# Autodesk Inventor assembly: ASY дренаж угольные
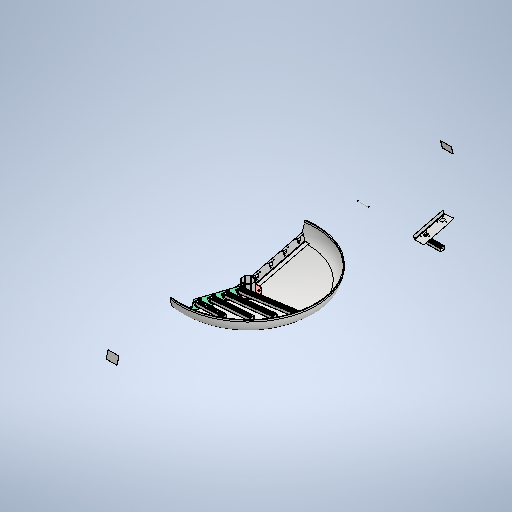
[picture p0: Inventor's stored thumbnail of the model, 512x512]
Saved by Autodesk Inventor 2025.1 (Build 291241020, 241B)
## iProperties
Created: 2024-12-09
Part Number: ASY дренаж угольные
Document SubType Name: Assembly
Designer: user
Author: user
## Documents named in this file (24)
- C:\Users\user\YandexDisk-badmisterfox\home pc\Inventor\filter-distribution-system\ASY BOTTOM filter distribution system.iam
- C:\Users\user\YandexDisk-badmisterfox\home pc\Inventor\filter-distribution-system\drain flange.ipt
- C:\Users\user\YandexDisk-badmisterfox\home pc\Inventor\filter-distribution-system\Фильтр напорный угольный 30 куб час.ipt
- C:\Users\user\YandexDisk-badmisterfox\home pc\Inventor\filter-distribution-system\MNT-CDF-501 box.ipt
- C:\Users\user\YandexDisk-badmisterfox\home pc\Inventor\filter-distribution-system\MNT-CDF-502 tube.ipt
- C:\Users\user\YandexDisk-badmisterfox\home pc\Inventor\filter-distribution-system\MNT-CDF-503  main tube 1.ipt
- C:\Users\user\YandexDisk-badmisterfox\home pc\Inventor\filter-distribution-system\MNT-CDF-504 small tube flange.ipt
- C:\Users\user\YandexDisk-badmisterfox\home pc\Inventor\filter-distribution-system\MNT-CDF-315 beam 5.ipt
- C:\Users\user\YandexDisk-badmisterfox\home pc\Inventor\filter-distribution-system\MNT-CDF-312 beam 2.ipt
- C:\Users\user\YandexDisk-badmisterfox\home pc\Inventor\filter-distribution-system\MNT-CDF-313 beam 3.ipt
- C:\Users\user\YandexDisk-badmisterfox\home pc\Inventor\filter-distribution-system\MNT-CDF-314 beam 4.ipt
- C:\Users\user\YandexDisk-badmisterfox\home pc\Inventor\filter-distribution-system\MNT-CDF-601 CAP.ipt
- C:\Users\user\YandexDisk-badmisterfox\home pc\Inventor\filter-distribution-system\MNT-CDF-602 CAP.ipt
- C:\Users\user\YandexDisk-badmisterfox\home pc\Inventor\filter-distribution-system\MNT-CDF-603 CAP.ipt
- C:\Users\user\YandexDisk-badmisterfox\home pc\Inventor\filter-distribution-system\ASY Луч 1.iam
- C:\Users\user\YandexDisk-badmisterfox\home pc\Inventor\filter-distribution-system\MNT-CDF-402 roof 875.ipt
- C:\Users\user\YandexDisk-badmisterfox\home pc\Inventor\filter-distribution-system\MNT-CDF-403 roof 775.ipt
- C:\Users\user\YandexDisk-badmisterfox\home pc\Inventor\filter-distribution-system\MNT-CDF-404 roof 675.ipt
- C:\Users\user\YandexDisk-badmisterfox\home pc\Inventor\filter-distribution-system\MNT-CDF-405 roof 475.ipt
- C:\Users\user\YandexDisk-badmisterfox\home pc\Inventor\filter-distribution-system\000 DS-B dimentions.ipt
- C:\Users\user\YandexDisk-badmisterfox\home pc\Inventor\filter-distribution-system\000 DS-B outer tube.ipt
- C:\Users\user\YandexDisk-badmisterfox\home pc\Inventor\filter-distribution-system\110 DS-B drain sustem flange.ipt
- C:\Users\user\YandexDisk-badmisterfox\home pc\Inventor\filter-distribution-system\MNT-CDF-613 big way.ipt
- C:\Users\user\YandexDisk-badmisterfox\home pc\Inventor\filter-distribution-system\MNT-CDF-604 CAP.ipt
## Components (34 placed, 23 different names)
1. 000 DS-B dimentions:1
2. Фильтр напорный угольный 30 куб час:1 — Mate:4, Flush:3, Flush:4, Rigid:36
3. MNT-CDF-501 box:1 — Mate:5, Flush:5, Mate:6, Rigid:40, Rigid:42, Rigid:43, Rigid:46, Rigid:47
4. drain flange:2 — Rigid:37
5. MNT-CDF-502 tube:4
6. MNT-CDF-502 tube:3
7. MNT-CDF-502 tube:2
8. MNT-CDF-503  main tube 1:1 — Rigid:39, Mate:7
9. MNT-CDF-503  main tube 1:2 — Mate:5, Rigid:38
10. MNT-CDF-501 box:2 — Mate:7, Mate:8, Mate:9
11. MNT-CDF-502 tube:5
12. MNT-CDF-405 roof 475:1 — Flush:15, Flush:16, Flush:17
13. MNT-CDF-315 beam 5:1 — Rigid:48, Flush:15, Flush:16, Flush:17
14. Part1:5 — Rigid:48
15. MNT-CDF-402 roof 875:1 — Flush:6, Flush:7, Flush:8
16. Part1:6 — Rigid:26, Rigid:43
17. MNT-CDF-604 CAP:1 — Rigid:44
18. MNT-CDF-312 beam 2:1 — Rigid:26, Flush:6, Flush:7, Flush:8, Rigid:44
19. Part1:7 — Rigid:27, Rigid:46
20. Part1:8 — Rigid:28, Rigid:47
21. MNT-CDF-313 beam 3:1 — Rigid:27, Flush:9, Flush:10, Flush:11, Rigid:45
22. MNT-CDF-403 roof 775:1 — Flush:9, Flush:10, Flush:11
23. MNT-CDF-404 roof 675:1 — Flush:12, Flush:13, Flush:14
24. MNT-CDF-314 beam 4:1 — Rigid:28, Flush:12, Flush:13, Flush:14
25. MNT-CDF-601 CAP:1
26. MNT-CDF-602 CAP:1
27. MNT-CDF-602 CAP:2
28. MNT-CDF-603 CAP:1 — Rigid:40, Rigid:41
29. MNT-CDF-603 CAP:2
30. ASY Луч 1:1 [sub-assembly] — Rigid:42
31. 000 DS-B outer tube:1 — Rigid:36, Rigid:37
32. drain sustem flange:1 — Mate:6, Rigid:38, Rigid:39, Mate:8
33. MNT-CDF-613 big way:1 — Rigid:41
34. MNT-CDF-604 CAP:2 — Rigid:45
## Relationships (37: WeldJoint 16, Flush 15, Mate 6)
- Mate:4: Фильтр напорный угольный 30 куб час:1
- Flush:3: Фильтр напорный угольный 30 куб час:1
- Flush:4: Фильтр напорный угольный 30 куб час:1
- Rigid:26 [WeldJoint]: Part1:6 ↔ MNT-CDF-312 beam 2:1
- Rigid:27 [WeldJoint]: Part1:7 ↔ MNT-CDF-313 beam 3:1
- Rigid:28 [WeldJoint]: Part1:8 ↔ MNT-CDF-314 beam 4:1
- Rigid:36 [WeldJoint]: Фильтр напорный угольный 30 куб час:1 ↔ 000 DS-B outer tube:1
- Rigid:37 [WeldJoint]: drain flange:2 ↔ 000 DS-B outer tube:1
- Mate:5: MNT-CDF-501 box:1 ↔ MNT-CDF-503  main tube 1:2
- Flush:5: MNT-CDF-501 box:1
- Mate:6: MNT-CDF-501 box:1 ↔ drain sustem flange:1
- Rigid:38 [WeldJoint]: MNT-CDF-503  main tube 1:2 ↔ drain sustem flange:1
- Rigid:39 [WeldJoint]: MNT-CDF-503  main tube 1:1 ↔ drain sustem flange:1
- Mate:7: MNT-CDF-503  main tube 1:1 ↔ MNT-CDF-501 box:2
- Mate:8: MNT-CDF-501 box:2 ↔ drain sustem flange:1
- Mate:9: MNT-CDF-501 box:2
- Rigid:40 [WeldJoint]: MNT-CDF-501 box:1 ↔ MNT-CDF-603 CAP:1
- Rigid:41 [WeldJoint]: MNT-CDF-603 CAP:1 ↔ MNT-CDF-613 big way:1
- Rigid:42 [WeldJoint]: MNT-CDF-501 box:1 ↔ ASY Луч 1:1
- Rigid:43 [WeldJoint]: MNT-CDF-501 box:1 ↔ Part1:6
- Flush:6: MNT-CDF-402 roof 875:1 ↔ MNT-CDF-312 beam 2:1
- Flush:7: MNT-CDF-402 roof 875:1 ↔ MNT-CDF-312 beam 2:1
- Flush:8: MNT-CDF-402 roof 875:1 ↔ MNT-CDF-312 beam 2:1
- Rigid:44 [WeldJoint]: MNT-CDF-604 CAP:1 ↔ MNT-CDF-312 beam 2:1
- Flush:9: MNT-CDF-313 beam 3:1 ↔ MNT-CDF-403 roof 775:1
- Flush:10: MNT-CDF-313 beam 3:1 ↔ MNT-CDF-403 roof 775:1
- Flush:11: MNT-CDF-313 beam 3:1 ↔ MNT-CDF-403 roof 775:1
- Rigid:45 [WeldJoint]: MNT-CDF-313 beam 3:1 ↔ MNT-CDF-604 CAP:2
- Rigid:46 [WeldJoint]: MNT-CDF-501 box:1 ↔ Part1:7
- Flush:12: MNT-CDF-404 roof 675:1 ↔ MNT-CDF-314 beam 4:1
- Flush:13: MNT-CDF-404 roof 675:1 ↔ MNT-CDF-314 beam 4:1
- Flush:14: MNT-CDF-404 roof 675:1 ↔ MNT-CDF-314 beam 4:1
- Rigid:47 [WeldJoint]: MNT-CDF-501 box:1 ↔ Part1:8
- Rigid:48 [WeldJoint]: MNT-CDF-315 beam 5:1 ↔ Part1:5
- Flush:15: MNT-CDF-405 roof 475:1 ↔ MNT-CDF-315 beam 5:1
- Flush:16: MNT-CDF-405 roof 475:1 ↔ MNT-CDF-315 beam 5:1
- Flush:17: MNT-CDF-405 roof 475:1 ↔ MNT-CDF-315 beam 5:1
